# Autodesk Inventor assembly: detectorArray
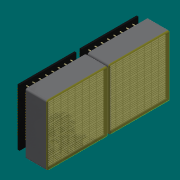
[picture p0: Inventor's stored thumbnail of the model, 180x180]
Saved by Autodesk Inventor 2016 SP1 (Build 200210100, 210)
## iProperties
Created: 2016-04-02
Part Number: detectorArray
Document SubType Name: Assembly
Designer: sawai
Author: sawai
## Documents named in this file (2)
- C:\Users\sawai\OneDrive\projects\modularRICH\detector\detectorArray.iam
- C:\Users\sawai\OneDrive\projects\modularRICH\dependency\H12700A\H12700A.iam
## Components (2 placed, 1 different names)
1. H12700A:1 [sub-assembly] — Flush:1, Flush:2, Mate:1
2. H12700A:2 [sub-assembly] — Flush:1, Flush:2, Mate:1
## Relationships (3: Flush 2, Mate 1)
- Flush:1: H12700A:1 ↔ H12700A:2
- Flush:2: H12700A:1 ↔ H12700A:2
- Mate:1 (1 mm): H12700A:1 ↔ H12700A:2
